# Autodesk Inventor assembly: wheel with drive motor floor
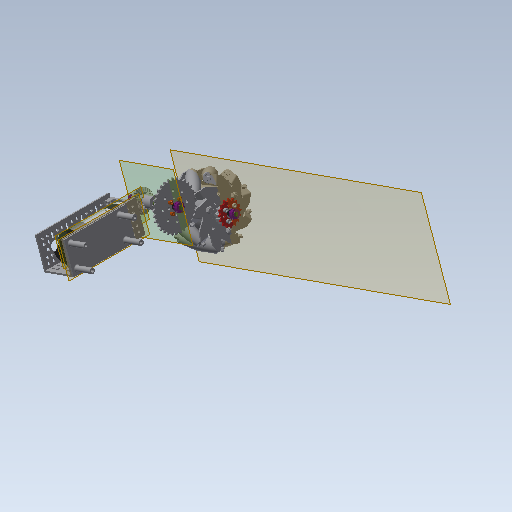
[picture p0: Inventor's stored thumbnail of the model, 512x512]
Saved by Autodesk Inventor 2020 (Build 240168000, 168)
## iProperties
Created: 2019-10-04
Part Number: wheel with drive motor floor
Document SubType Name: Assembly
Designer: ball
Author: ball
## Documents named in this file (6)
- D:\FTC8863\2019 Robot\Mecanum Drive Train\wheel with drive motor top.iam
- D:\FTC8863\2019 Robot\Mecanum Drive Train\motor with bevil gear and sprocket.iam
- D:\FTC8863\2019 Robot\Mecanum Drive Train\wheel with sprocket.iam
- D:\FTC8863\GoBilda\1120 Parts\1120-0004-0120.ipt
- D:\FTC8863\GoBilda\1702 Parts\1702-0032-0002 assembly.ipt
- D:\FTC8863\2019 Robot\Mecanum Drive Train\spacer for new drivetrain 2.ipt
## Components (5 placed, 5 different names)
1. motor with bevil gear and sprocket:1 [sub-assembly] — Flush:2, Flush:3, Mate:1, Mate:2, Mate:5, Angle:2
2. wheel with sprocket:1 [sub-assembly] — Flush:2, Flush:3, Mate:5
3. 1120-0004-0120:1 — Mate:3, Mate:4, Angle:1, Angle:2, Flush:4, Flush:5
4. 1702-0032-0002 assembly:1 — Mate:1, Mate:2, Mate:3, Mate:4, Angle:1
5. spacer for new drivetrain 2:1 — Flush:4, Flush:5
## Relationships (11: Mate 5, Flush 4, Angle 2)
- Flush:2 (-43.18 mm): motor with bevil gear and sprocket:1 ↔ wheel with sprocket:1
- Flush:3: motor with bevil gear and sprocket:1 ↔ wheel with sprocket:1
- Mate:1: motor with bevil gear and sprocket:1 ↔ 1702-0032-0002 assembly:1
- Mate:2: motor with bevil gear and sprocket:1 ↔ 1702-0032-0002 assembly:1
- Mate:3: 1120-0004-0120:1 ↔ 1702-0032-0002 assembly:1
- Mate:4: 1120-0004-0120:1 ↔ 1702-0032-0002 assembly:1
- Angle:1 (0 deg): 1120-0004-0120:1 ↔ 1702-0032-0002 assembly:1
- Mate:5 (76.2 mm): motor with bevil gear and sprocket:1 ↔ wheel with sprocket:1
- Angle:2 (180 deg): motor with bevil gear and sprocket:1 ↔ 1120-0004-0120:1
- Flush:4: 1120-0004-0120:1 ↔ spacer for new drivetrain 2:1
- Flush:5: 1120-0004-0120:1 ↔ spacer for new drivetrain 2:1
